# Autodesk Inventor assembly: Z_galvo_optosigma_assembly
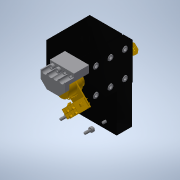
[picture p0: Inventor's stored thumbnail of the model, 180x180]
Saved by Autodesk Inventor 2022 (Build 260153000, 153)
## iProperties
Created: 2018-06-13
Part Number: Z_galvo_optosigma_assembly
Document SubType Name: Assembly
Designer: legant_local
Author: legant_local
## Documents named in this file (13)
- G:\My Drive\OPM\2P-OPM_CAD\workspace\Sub-assemblies\Z_galvo_optosigma_assembly.iam
- G:\My Drive\OPM\2P-OPM_CAD\workspace\Imported Components\Cambridge_Technology\D05893 w_D07861.ipt
- G:\My Drive\OPM\2P-OPM_CAD\workspace\Imported Components\OptoSigma\TADC-251SR.iam
- G:\My Drive\OPM\2P-OPM_CAD\workspace\Imported Components\McMaster_Carr\McMaster_Carr_91292A014_M2p5x10mm_socket_cap.ipt
- G:\My Drive\OPM\2P-OPM_CAD\workspace\Imported Components\McMaster_Carr\McMaster_Carr_92290A012_M2x5mm_socket_cap.ipt
- G:\My Drive\OPM\2P-OPM_CAD\workspace\Imported Components\McMaster_Carr\McMaster_Carr_92290A017_M2x10mm_socket_cap.ipt
- G:\My Drive\OPM\2P-OPM_CAD\workspace\Imported Components\McMaster_Carr\McMaster_Carr_91292A833_M2x10mm_socket_cap.ipt
- E:\AOLLS_SVN\workspace\Imported Components\McMaster_Carr\McMaster_Carr_91595A019_METRIC ALLOY STEEL DOWEL PIN_D2_L5.ipt
- G:\My Drive\OPM\2P-OPM_CAD\workspace\Imported Components\McMaster_Carr\McMaster_Carr_92290A746_M2x16mm_socket_cap.ipt
- G:\My Drive\OPM\2P-OPM_CAD\workspace\Custom Parts Linked With Drawings\xgalvo_to_base_clamp.ipt
- G:\My Drive\OPM\2P-OPM_CAD\workspace\Custom Parts Linked With Drawings\zgalvo_to_optisigma_stage.ipt
- G:\My Drive\OPM\2P-OPM_CAD\workspace\Custom 3D Printed Parts\galvo_stop.ipt
- G:\My Drive\OPM\2P-OPM_CAD\workspace\Custom 3D Printed Parts\zgalvo_cover.ipt
## Components (30 placed, 12 different names)
1. D05893 w_D07861:1 — Mate:1, Angle:1, Mate:6
2. zgalvo_to_optisigma_stage:1 — Mate:1, Mate:2, Angle:1, Mate:22, Mate:23, Mate:24, Mate:25, Mate:26, Mate:27, Flush:12, Mate:39, Mate:40, Mate:41, Mate:42, Mate:43, Mate:48, Mate:49, Mate:50, Mate:55, Mate:56
3. McMaster_Carr_91595A019_METRIC ALLOY STEEL DOWEL PIN_D2_L5:1 — Tangent:2, Mate:48
4. McMaster_Carr_91595A019_METRIC ALLOY STEEL DOWEL PIN_D2_L5:2 — Tangent:1, Mate:50
5. McMaster_Carr_91595A019_METRIC ALLOY STEEL DOWEL PIN_D2_L5:3 — Tangent:3, Mate:49
6. TADC-251SR:1 [sub-assembly] — Mate:2, Tangent:1, Tangent:2, Tangent:3, Mate:6, Tangent:4, Tangent:5, Tangent:6, Mate:17, Mate:18, Mate:19, Mate:20, Mate:21, Mate:51, Mate:52, Mate:53
7. McMaster_Carr_91595A019_METRIC ALLOY STEEL DOWEL PIN_D2_L5:4 — Tangent:4, Mate:52
8. McMaster_Carr_91595A019_METRIC ALLOY STEEL DOWEL PIN_D2_L5:5 — Tangent:5, Mate:53
9. McMaster_Carr_91595A019_METRIC ALLOY STEEL DOWEL PIN_D2_L5:6 — Tangent:6, Mate:51
10. McMaster_Carr_91292A014_M2p5x10mm_socket_cap:1 — Flush:4, Flush:5, Mate:13, Mate:16, Flush:13, Flush:14, Flush:15
11. McMaster_Carr_91292A014_M2p5x10mm_socket_cap:2 — Flush:4, Mate:14
12. McMaster_Carr_91292A014_M2p5x10mm_socket_cap:3 — Flush:5, Mate:15
13. McMaster_Carr_92290A012_M2x5mm_socket_cap:1 — Flush:6, Flush:7, Flush:8, Mate:20
14. McMaster_Carr_92290A012_M2x5mm_socket_cap:2 — Flush:6, Mate:17, Mate:21
15. McMaster_Carr_92290A012_M2x5mm_socket_cap:3 — Flush:7, Mate:19
16. McMaster_Carr_92290A012_M2x5mm_socket_cap:4 — Flush:8, Mate:18
17. McMaster_Carr_92290A017_M2x10mm_socket_cap:1 — Flush:9, Flush:10, Flush:11, Mate:22
18. McMaster_Carr_92290A017_M2x10mm_socket_cap:2 — Flush:9, Mate:25, Mate:26
19. McMaster_Carr_92290A017_M2x10mm_socket_cap:3 — Flush:10, Mate:24
20. McMaster_Carr_92290A017_M2x10mm_socket_cap:4 — Flush:11, Mate:23
21. xgalvo_to_base_clamp:1 — Mate:27, Flush:12, Mate:13, Mate:14, Mate:15, Mate:28, Mate:29, Mate:30, Mate:16, Mate:40
22. McMaster_Carr_91292A014_M2p5x10mm_socket_cap:4 — Flush:13, Mate:28
23. McMaster_Carr_91292A014_M2p5x10mm_socket_cap:5 — Flush:14, Mate:29
24. McMaster_Carr_91292A014_M2p5x10mm_socket_cap:6 — Flush:15, Mate:30
25. galvo_stop:1 — Mate:39, Mate:54, Mate:55, Mate:56, Mate:57, Mate:58
26. McMaster_Carr_92290A746_M2x16mm_socket_cap:1 — Mate:54, Mate:57
27. McMaster_Carr_92290A746_M2x16mm_socket_cap:2 — Mate:58
28. zgalvo_cover:1 — Mate:41, Mate:42, Mate:43, Mate:44, Mate:45, Mate:46, Mate:47
29. McMaster_Carr_91292A833_M2x10mm_socket_cap:1 — Mate:44, Mate:46
30. McMaster_Carr_91292A833_M2x10mm_socket_cap:2 — Mate:45, Mate:47
## Relationships (67: Mate 48, Flush 12, Tangent 6, Angle 1)
- Mate:1: D05893 w_D07861:1 ↔ zgalvo_to_optisigma_stage:1
- Mate:2: zgalvo_to_optisigma_stage:1 ↔ TADC-251SR:1
- [Mate]: zgalvo_to_optisigma_stage:1 ↔ McMaster_Carr_91595A019_METRIC ALLOY STEEL DOWEL PIN_D2_L5:1
- [Mate]: zgalvo_to_optisigma_stage:1 ↔ McMaster_Carr_91595A019_METRIC ALLOY STEEL DOWEL PIN_D2_L5:2
- [Mate]: zgalvo_to_optisigma_stage:1 ↔ McMaster_Carr_91595A019_METRIC ALLOY STEEL DOWEL PIN_D2_L5:3
- Tangent:1: McMaster_Carr_91595A019_METRIC ALLOY STEEL DOWEL PIN_D2_L5:2 ↔ TADC-251SR:1
- Tangent:2: McMaster_Carr_91595A019_METRIC ALLOY STEEL DOWEL PIN_D2_L5:1 ↔ TADC-251SR:1
- Tangent:3: McMaster_Carr_91595A019_METRIC ALLOY STEEL DOWEL PIN_D2_L5:3 ↔ TADC-251SR:1
- Angle:1 (225 deg): D05893 w_D07861:1 ↔ zgalvo_to_optisigma_stage:1
- Mate:6 (-35 mm): D05893 w_D07861:1 ↔ TADC-251SR:1
- Tangent:4: TADC-251SR:1 ↔ McMaster_Carr_91595A019_METRIC ALLOY STEEL DOWEL PIN_D2_L5:4
- Tangent:5: TADC-251SR:1 ↔ McMaster_Carr_91595A019_METRIC ALLOY STEEL DOWEL PIN_D2_L5:5
- Tangent:6: TADC-251SR:1 ↔ McMaster_Carr_91595A019_METRIC ALLOY STEEL DOWEL PIN_D2_L5:6
- [Mate] (-5 mm): TADC-251SR:1 ↔ McMaster_Carr_91595A019_METRIC ALLOY STEEL DOWEL PIN_D2_L5:4
- [Mate] (-5 mm): TADC-251SR:1 ↔ McMaster_Carr_91595A019_METRIC ALLOY STEEL DOWEL PIN_D2_L5:5
- [Mate] (-2 mm): TADC-251SR:1 ↔ McMaster_Carr_91595A019_METRIC ALLOY STEEL DOWEL PIN_D2_L5:6
- Flush:4: McMaster_Carr_91292A014_M2p5x10mm_socket_cap:1 ↔ McMaster_Carr_91292A014_M2p5x10mm_socket_cap:2
- Flush:5: McMaster_Carr_91292A014_M2p5x10mm_socket_cap:1 ↔ McMaster_Carr_91292A014_M2p5x10mm_socket_cap:3
- Mate:13: McMaster_Carr_91292A014_M2p5x10mm_socket_cap:1 ↔ xgalvo_to_base_clamp:1
- Mate:14: McMaster_Carr_91292A014_M2p5x10mm_socket_cap:2 ↔ xgalvo_to_base_clamp:1
- Mate:15: McMaster_Carr_91292A014_M2p5x10mm_socket_cap:3 ↔ xgalvo_to_base_clamp:1
- Mate:16: McMaster_Carr_91292A014_M2p5x10mm_socket_cap:1 ↔ xgalvo_to_base_clamp:1
- Flush:6: McMaster_Carr_92290A012_M2x5mm_socket_cap:1 ↔ McMaster_Carr_92290A012_M2x5mm_socket_cap:2
- Flush:7: McMaster_Carr_92290A012_M2x5mm_socket_cap:1 ↔ McMaster_Carr_92290A012_M2x5mm_socket_cap:3
- Flush:8: McMaster_Carr_92290A012_M2x5mm_socket_cap:1 ↔ McMaster_Carr_92290A012_M2x5mm_socket_cap:4
- Mate:17: TADC-251SR:1 ↔ McMaster_Carr_92290A012_M2x5mm_socket_cap:2
- Mate:18: TADC-251SR:1 ↔ McMaster_Carr_92290A012_M2x5mm_socket_cap:4
- Mate:19: TADC-251SR:1 ↔ McMaster_Carr_92290A012_M2x5mm_socket_cap:3
- Mate:20: TADC-251SR:1 ↔ McMaster_Carr_92290A012_M2x5mm_socket_cap:1
- Mate:21: TADC-251SR:1 ↔ McMaster_Carr_92290A012_M2x5mm_socket_cap:2
- Flush:9: McMaster_Carr_92290A017_M2x10mm_socket_cap:1 ↔ McMaster_Carr_92290A017_M2x10mm_socket_cap:2
- Flush:10: McMaster_Carr_92290A017_M2x10mm_socket_cap:1 ↔ McMaster_Carr_92290A017_M2x10mm_socket_cap:3
- Flush:11: McMaster_Carr_92290A017_M2x10mm_socket_cap:1 ↔ McMaster_Carr_92290A017_M2x10mm_socket_cap:4
- Mate:22: zgalvo_to_optisigma_stage:1 ↔ McMaster_Carr_92290A017_M2x10mm_socket_cap:1
- Mate:23: zgalvo_to_optisigma_stage:1 ↔ McMaster_Carr_92290A017_M2x10mm_socket_cap:4
- Mate:24: zgalvo_to_optisigma_stage:1 ↔ McMaster_Carr_92290A017_M2x10mm_socket_cap:3
- Mate:25: zgalvo_to_optisigma_stage:1 ↔ McMaster_Carr_92290A017_M2x10mm_socket_cap:2
- Mate:26: zgalvo_to_optisigma_stage:1 ↔ McMaster_Carr_92290A017_M2x10mm_socket_cap:2
- Mate:27: zgalvo_to_optisigma_stage:1 ↔ xgalvo_to_base_clamp:1
- Flush:12: zgalvo_to_optisigma_stage:1 ↔ xgalvo_to_base_clamp:1
- Flush:13: McMaster_Carr_91292A014_M2p5x10mm_socket_cap:1 ↔ McMaster_Carr_91292A014_M2p5x10mm_socket_cap:4
- Flush:14: McMaster_Carr_91292A014_M2p5x10mm_socket_cap:1 ↔ McMaster_Carr_91292A014_M2p5x10mm_socket_cap:5
- Flush:15: McMaster_Carr_91292A014_M2p5x10mm_socket_cap:1 ↔ McMaster_Carr_91292A014_M2p5x10mm_socket_cap:6
- Mate:28: xgalvo_to_base_clamp:1 ↔ McMaster_Carr_91292A014_M2p5x10mm_socket_cap:4
- Mate:29: xgalvo_to_base_clamp:1 ↔ McMaster_Carr_91292A014_M2p5x10mm_socket_cap:5
- Mate:30: xgalvo_to_base_clamp:1 ↔ McMaster_Carr_91292A014_M2p5x10mm_socket_cap:6
- [Mate]: galvo_stop:1 ↔ McMaster_Carr_92290A746_M2x16mm_socket_cap:2
- Mate:39: zgalvo_to_optisigma_stage:1 ↔ galvo_stop:1
- Mate:40: zgalvo_to_optisigma_stage:1 ↔ xgalvo_to_base_clamp:1
- Mate:41: zgalvo_to_optisigma_stage:1 ↔ zgalvo_cover:1
- Mate:42: zgalvo_to_optisigma_stage:1 ↔ zgalvo_cover:1
- Mate:43: zgalvo_to_optisigma_stage:1 ↔ zgalvo_cover:1
- Mate:44: zgalvo_cover:1 ↔ McMaster_Carr_91292A833_M2x10mm_socket_cap:1
- Mate:45: zgalvo_cover:1 ↔ McMaster_Carr_91292A833_M2x10mm_socket_cap:2
- Mate:46: zgalvo_cover:1 ↔ McMaster_Carr_91292A833_M2x10mm_socket_cap:1
- Mate:47: zgalvo_cover:1 ↔ McMaster_Carr_91292A833_M2x10mm_socket_cap:2
- Mate:48 (2 mm): zgalvo_to_optisigma_stage:1 ↔ McMaster_Carr_91595A019_METRIC ALLOY STEEL DOWEL PIN_D2_L5:1
- Mate:49 (2 mm): zgalvo_to_optisigma_stage:1 ↔ McMaster_Carr_91595A019_METRIC ALLOY STEEL DOWEL PIN_D2_L5:3
- Mate:50 (2 mm): zgalvo_to_optisigma_stage:1 ↔ McMaster_Carr_91595A019_METRIC ALLOY STEEL DOWEL PIN_D2_L5:2
- Mate:51 (-2 mm): TADC-251SR:1 ↔ McMaster_Carr_91595A019_METRIC ALLOY STEEL DOWEL PIN_D2_L5:6
- Mate:52 (-2 mm): TADC-251SR:1 ↔ McMaster_Carr_91595A019_METRIC ALLOY STEEL DOWEL PIN_D2_L5:4
- Mate:53 (-2 mm): TADC-251SR:1 ↔ McMaster_Carr_91595A019_METRIC ALLOY STEEL DOWEL PIN_D2_L5:5
- Mate:54: galvo_stop:1 ↔ McMaster_Carr_92290A746_M2x16mm_socket_cap:1
- Mate:55: zgalvo_to_optisigma_stage:1 ↔ galvo_stop:1
- Mate:56: zgalvo_to_optisigma_stage:1 ↔ galvo_stop:1
- Mate:57: galvo_stop:1 ↔ McMaster_Carr_92290A746_M2x16mm_socket_cap:1
- Mate:58: galvo_stop:1 ↔ McMaster_Carr_92290A746_M2x16mm_socket_cap:2
## Named parameters: d61_d34 = 0 mm
